# Autodesk Inventor assembly: Table
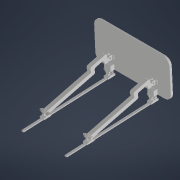
[picture p0: Inventor's stored thumbnail of the model, 180x180]
Saved by Autodesk Inventor 2021 (Build 250183000, 183)
## iProperties
Created: 2021-01-30
Part Number: Table
Document SubType Name: Assembly
Designer: PaisW
Author: PaisW
## Documents named in this file (7)
- C:\Users\argon\OneDrive\Documents\GrabCAD\EngOne Maroons\Table Subassemly\Table Subassembly.iam
- C:\Users\argon\OneDrive\Documents\GrabCAD\EngOne Maroons\Table Subassemly\Table Post\Guide Rail.ipt
- C:\Users\argon\OneDrive\Documents\GrabCAD\EngOne Maroons\Table Subassemly\Tabletop\Table.ipt
- C:\Users\argon\OneDrive\Documents\GrabCAD\EngOne Maroons\Table Subassemly\HingeSubassembly.iam
- C:\Users\argon\OneDrive\Documents\GrabCAD\EngOne Maroons\Table Subassemly\WirelessChargerBase.ipt
- C:\Users\argon\OneDrive\Documents\GrabCAD\EngOne Maroons\Table Subassemly\Table Post\DoubleHinge.ipt
- C:\Users\argon\OneDrive\Documents\GrabCAD\EngOne Maroons\Table Subassemly\Table Post\Support.ipt
## Components (14 placed, 6 different names)
1. Guide Rail:1 — Flush:7, Mate:26, Mate:27, Flush:8, Flush:9, Mate:32, Mate:34
2. Guide Rail:2 — Flush:7, Mate:28, Mate:29, Flush:8, Flush:9, Mate:31, Mate:33, Flush:10, Flush:11
3. Table:1 — Mate:36, Mate:37, Mate:38, Mate:39, Mate:40, Mate:41, Mate:42, Mate:43, Mate:44, Mate:45, Mate:46, Mate:47, Mate:48, Mate:49, Angle:1, Angle:2
4. HingeSubassembly:1 [sub-assembly] — Mate:31, Mate:33, Mate:35, Mate:53, Mate:54, Flush:11
5. HingeSubassembly:2 [sub-assembly] — Mate:26, Mate:27, Mate:30, Mate:52
6. HingeSubassembly:3 [sub-assembly] — Mate:32, Mate:34, Mate:35, Mate:55, Mate:56
7. HingeSubassembly:4 [sub-assembly] — Mate:28, Mate:29, Mate:30, Mate:50, Mate:51, Flush:10, Angle:2
8. WirelessChargerBase:1 — Mate:36, Mate:37, Angle:1
9. DoubleHinge:1 — Mate:38, Mate:39, Mate:40, Mate:58
10. DoubleHinge:2 — Mate:41, Mate:42, Mate:43, Mate:57
11. DoubleHinge:3 — Mate:47, Mate:48, Mate:49, Mate:50, Mate:51
12. DoubleHinge:4 — Mate:44, Mate:45, Mate:46, Mate:52
13. Support:1 — Mate:53, Mate:54, Mate:57
14. Support:2 — Mate:55, Mate:56, Mate:58
## Relationships (40: Mate 33, Flush 5, Angle 2)
- Flush:7: Guide Rail:1 ↔ Guide Rail:2
- Mate:26: Guide Rail:1 ↔ HingeSubassembly:2
- Mate:27: Guide Rail:1 ↔ HingeSubassembly:2
- Mate:28: Guide Rail:2 ↔ HingeSubassembly:4
- Mate:29: Guide Rail:2 ↔ HingeSubassembly:4
- Flush:8: Guide Rail:1 ↔ Guide Rail:2
- Flush:9: Guide Rail:1 ↔ Guide Rail:2
- Mate:30: HingeSubassembly:2 ↔ HingeSubassembly:4
- Mate:31: Guide Rail:2 ↔ HingeSubassembly:1
- Mate:32: Guide Rail:1 ↔ HingeSubassembly:3
- Mate:33: Guide Rail:2 ↔ HingeSubassembly:1
- Mate:34: Guide Rail:1 ↔ HingeSubassembly:3
- Mate:35: HingeSubassembly:1 ↔ HingeSubassembly:3
- Mate:36: Table:1 ↔ WirelessChargerBase:1
- Mate:37: Table:1 ↔ WirelessChargerBase:1
- Mate:38: Table:1 ↔ DoubleHinge:1
- Mate:39: Table:1 ↔ DoubleHinge:1
- Mate:40: Table:1 ↔ DoubleHinge:1
- Mate:41: Table:1 ↔ DoubleHinge:2
- Mate:42: Table:1 ↔ DoubleHinge:2
- Mate:43: Table:1 ↔ DoubleHinge:2
- Mate:44: Table:1 ↔ DoubleHinge:4
- Mate:45: Table:1 ↔ DoubleHinge:4
- Mate:46: Table:1 ↔ DoubleHinge:4
- Mate:47: Table:1 ↔ DoubleHinge:3
- Mate:48: Table:1 ↔ DoubleHinge:3
- Mate:49: Table:1 ↔ DoubleHinge:3
- Mate:50: HingeSubassembly:4 ↔ DoubleHinge:3
- Mate:51: HingeSubassembly:4 ↔ DoubleHinge:3
- Mate:52: HingeSubassembly:2 ↔ DoubleHinge:4
- Mate:53: HingeSubassembly:1 ↔ Support:1
- Mate:54: HingeSubassembly:1 ↔ Support:1
- Mate:55: HingeSubassembly:3 ↔ Support:2
- Mate:56: HingeSubassembly:3 ↔ Support:2
- Mate:57: DoubleHinge:2 ↔ Support:1
- Mate:58: DoubleHinge:1 ↔ Support:2
- Angle:1 (-180 deg): Table:1 ↔ WirelessChargerBase:1
- Flush:10: Guide Rail:2 ↔ HingeSubassembly:4
- Angle:2 (-90 deg): Table:1 ↔ HingeSubassembly:4
- Flush:11: Guide Rail:2 ↔ HingeSubassembly:1
